# Autodesk Inventor assembly: RailAttachmentAssembly
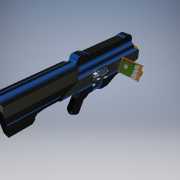
[picture p0: Inventor's stored thumbnail of the model, 180x180]
Saved by Autodesk Inventor 2018 (Build 220112000, 112)
## iProperties
Created: 2019-04-01
Part Number: RailAttachmentAssembly
Document SubType Name: Assembly
Designer: snipe
Author: snipe
## Documents named in this file (4)
- C:\Users\snipe\Documents\CPRE186-CAD\RailAttachmentAssemblyWithGun.iam
- C:\Users\snipe\Documents\CPRE186-CAD\NerfRivalZeus.ipt
- C:\Users\snipe\Documents\CPRE186-CAD\ArduinoUno.iam
- C:\Users\snipe\Documents\CPRE186-CAD\RailAttachmentAssemblyLeft.iam
## Components (3 placed, 3 different names)
1. NerfRivalZeus:1 — Mate:2, Mate:1, Mate:3, Mate:5, Mate:6
2. ArduinoUno:1 [sub-assembly] — Mate:6
3. RailAttachmentAssemblyLeft:1 [sub-assembly] — Mate:5
## Relationships (5: Mate 5)
- Mate:2: NerfRivalZeus:1
- Mate:1: NerfRivalZeus:1
- Mate:3: NerfRivalZeus:1
- Mate:5: NerfRivalZeus:1 ↔ RailAttachmentAssemblyLeft:1
- Mate:6: NerfRivalZeus:1 ↔ ArduinoUno:1
